# Autodesk Inventor assembly: kicker_assembly_v2
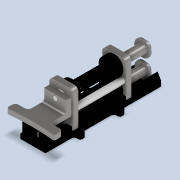
[picture p0: Inventor's stored thumbnail of the model, 180x180]
Saved by Autodesk Inventor 2020.4 (Build 244396000, 396)
## iProperties
Created: 2019-08-27
Part Number: kicker_assembly_v2
Document SubType Name: Assembly
Designer: felip
Author: felip
## Documents named in this file (10)
- G:\Meu Drive\RobôCIn\Mecânica\SSL\2021\Inventor\first_floor\Kicker\kicker_assembly.iam
- G:\Meu Drive\RobôCIn\Mecânica\SSL\2021\Inventor\first_floor\Kicker\kicker_base.ipt
- G:\Meu Drive\RobôCIn\Mecânica\SSL\2021\Inventor\first_floor\Kicker\kicker_assembly_chip.iam
- G:\Meu Drive\RobôCIn\Mecânica\SSL\2021\Inventor\first_floor\Kicker\kicker_assembly_front.iam
- G:\Meu Drive\RobôCIn\Mecânica\SSL\2021\Inventor\first_floor\Kicker\compras\ScrewM3x12.ipt
- G:\Meu Drive\RobôCIn\Mecânica\SSL\2021\Inventor\first_floor\Kicker\compras\Wurth 963040042.ipt
- G:\Meu Drive\RobôCIn\Mecânica\SSL\2021\Inventor\first_floor\Kicker\compras\Wurth 970500361.ipt
- G:\Meu Drive\RobôCIn\Mecânica\SSL\2021\Inventor\first_floor\Kicker\kicker_coil_front.ipt
- G:\Meu Drive\RobôCIn\Mecânica\SSL\2021\Inventor\first_floor\Kicker\kicker_coil_chip.ipt
- G:\Meu Drive\RobôCIn\Mecânica\SSL\2021\Inventor\first_floor\Kicker\kicker_plate_modified.ipt
## Components (15 placed, 9 different names)
1. Kicker Base:1 — Rigid:11, Rigid:12, Cylindrical:2, Cylindrical:3, Mate:7, Mate:8, Mate:9, Mate:10, Mate:11
2. Kicker Base:2 — Rigid:3, Rigid:7, Rigid:8, Rigid:9, Rigid:10
3. Kicker Coil Chip:1 — Rigid:3
4. Kicker Coil Front:1
5. Kicker Chip Assembly:1 [sub-assembly] — Cylindrical:3, Mate:8
6. Kicker Front Assembly:1 [sub-assembly] — Cylindrical:2, Mate:7
7. ScrewM3x12:1 — Rigid:11
8. ScrewM3x12:2 — Rigid:12
9. ScrewM3x12:3 — Rigid:10
10. ScrewM3x12:4 — Rigid:9
11. Wurth 963040042:1 — Rigid:5, Rigid:7
12. Wurth 963040042:2 — Rigid:6, Rigid:8
13. Wurth 970500361:1 — Rigid:5
14. Wurth 970500361:2 — Rigid:6
15. Kicker Plate:1 — Mate:9, Mate:10, Mate:11
## Relationships (16: WeldJoint 9, Mate 5, CylindricalJoint 2)
- Rigid:3 [WeldJoint]: Kicker Base:2 ↔ Kicker Coil Chip:1
- Rigid:5 [WeldJoint]: Wurth 963040042:1 ↔ Wurth 970500361:1
- Rigid:6 [WeldJoint]: Wurth 963040042:2 ↔ Wurth 970500361:2
- Rigid:7 [WeldJoint]: Kicker Base:2 ↔ Wurth 963040042:1
- Rigid:8 [WeldJoint]: Kicker Base:2 ↔ Wurth 963040042:2
- Rigid:9 [WeldJoint]: Kicker Base:2 ↔ ScrewM3x12:4
- Rigid:10 [WeldJoint]: Kicker Base:2 ↔ ScrewM3x12:3
- Rigid:11 [WeldJoint]: Kicker Base:1 ↔ ScrewM3x12:1
- Rigid:12 [WeldJoint]: Kicker Base:1 ↔ ScrewM3x12:2
- Cylindrical:2: Kicker Base:1 ↔ Kicker Front Assembly:1
- Cylindrical:3: Kicker Base:1 ↔ Kicker Chip Assembly:1
- Mate:7 (1 mm): Kicker Base:1 ↔ Kicker Front Assembly:1
- Mate:8 (1 mm): Kicker Base:1 ↔ Kicker Chip Assembly:1
- Mate:9: Kicker Base:1 ↔ Kicker Plate:1
- Mate:10: Kicker Base:1 ↔ Kicker Plate:1
- Mate:11: Kicker Base:1 ↔ Kicker Plate:1
